# Autodesk Inventor assembly: Assembly7
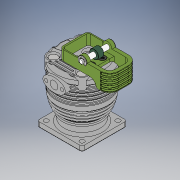
[picture p0: Inventor's stored thumbnail of the model, 180x180]
Saved by Autodesk Inventor 2018 (Build 220112000, 112)
## iProperties
Created: 2023-04-25
Part Number: Assembly7
Document SubType Name: Assembly
Designer: Habib Mohamed
Author: Habib Mohamed
## Documents named in this file (13)
- D:\Inventor\My projects\Rotary Engine\Assembly\Assembly7.iam
- Cykinder SubAssembly.iam
- D:\Inventor\My projects\Rotary Engine\Component 13 (Cylinder Liner).ipt
- D:\Inventor\My projects\Rotary Engine\Component 22 (Cylinder Base Gasket).ipt
- D:\Inventor\My projects\Rotary Engine\Component 35(Cylinder Top Gasket).ipt
- D:\Inventor\My projects\Rotary Engine\Component 50(Cylinder Head).ipt
- D:\Inventor\My projects\Rotary Engine\Component 49(Cylinder).ipt
- D:\Inventor\My projects\Rotary Engine\Component 25 (Rocker Arm Axle).ipt
- D:\Inventor\My projects\Rotary Engine\Component 36(Rocker Arm Bracket).ipt
- D:\Inventor\My projects\Rotary Engine\Component 14 (Spacer Sleeve).ipt
- C:\Users\Habib Mohamed\Documents\Inventor\Content Center Files\R2018\en-US\DIN EN ISO 4014\DIN EN ISO 4014 - M4 x 25.ipt
- C:\Users\Habib Mohamed\Documents\Inventor\Content Center Files\R2018\en-US\ISO 7046-1 Z(1)\ISO 7046-1 - M3 x 10 - 4.8 - Z - ISO.ipt
- C:\Users\Habib Mohamed\Documents\Inventor\Content Center Files\R2018\en-US\DIN 6799\DIN 6799 - 3.2 4.ipt
## Components (16 placed, 11 different names)
1. Component 13 (Cylinder Liner):1 — Mate:7, Mate:8, Mate:9, Mate:12
2. Component 22 (Cylinder Base Gasket):1 — Mate:11, Mate:12, Mate:13
3. Component 35(Cylinder Top Gasket):1 — Mate:6, Mate:9
4. Component 50(Cylinder Head):1 — Mate:4, Mate:5, Mate:10, Mate:15, Mate:17, Mate:19, Mate:21, Mate:22, Mate:23, Mate:24
5. Component 49(Cylinder):1 — Mate:1, Mate:2, Mate:3, Mate:4, Mate:5, Mate:6, Mate:7, Mate:8, Mate:10, Mate:11, Mate:13, Mate:14, Mate:16, Mate:18, Mate:20
6. Component 25 (Rocker Arm Axle):1 — Mate:25, Mate:26, Mate:27, Mate:31, Mate:33
7. Component 36(Rocker Arm Bracket):1 — Mate:22, Mate:23, Mate:24, Mate:26, Mate:27, Mate:28, Mate:29, Mate:30, Mate:32, Mate:34
8. Component 14 (Spacer Sleeve):1 — Mate:25, Mate:28
9. DIN EN ISO 4014 M4 x 25:1 — Mate:14, Mate:15
10. DIN EN ISO 4014 M4 x 25:2 — Mate:16, Mate:17
11. DIN EN ISO 4014 M4 x 25:3 — Mate:18, Mate:19
12. DIN EN ISO 4014 M4 x 25:4 — Mate:20, Mate:21
13. ISO 7046-1 Z M3 x 10 - 4.8 - Z:1 — Mate:29
14. ISO 7046-1 Z M3 x 10 - 4.8 - Z:2 — Mate:30
15. DIN 6799 3.2:1 — Mate:31, Mate:32
16. DIN 6799 3.2:2 — Mate:33, Mate:34
## Relationships (34: Mate 34)
- Mate:1: Component 49(Cylinder):1
- Mate:2: Component 49(Cylinder):1
- Mate:3: Component 49(Cylinder):1
- Mate:4: Component 50(Cylinder Head):1 ↔ Component 49(Cylinder):1
- Mate:5: Component 50(Cylinder Head):1 ↔ Component 49(Cylinder):1
- Mate:6: Component 35(Cylinder Top Gasket):1 ↔ Component 49(Cylinder):1
- Mate:7: Component 13 (Cylinder Liner):1 ↔ Component 49(Cylinder):1
- Mate:8: Component 13 (Cylinder Liner):1 ↔ Component 49(Cylinder):1
- Mate:9: Component 13 (Cylinder Liner):1 ↔ Component 35(Cylinder Top Gasket):1
- Mate:10: Component 50(Cylinder Head):1 ↔ Component 49(Cylinder):1
- Mate:11: Component 22 (Cylinder Base Gasket):1 ↔ Component 49(Cylinder):1
- Mate:12: Component 13 (Cylinder Liner):1 ↔ Component 22 (Cylinder Base Gasket):1
- Mate:13: Component 22 (Cylinder Base Gasket):1 ↔ Component 49(Cylinder):1
- Mate:14: Component 49(Cylinder):1 ↔ DIN EN ISO 4014 M4 x 25:1
- Mate:15: Component 50(Cylinder Head):1 ↔ DIN EN ISO 4014 M4 x 25:1
- Mate:16: Component 49(Cylinder):1 ↔ DIN EN ISO 4014 M4 x 25:2
- Mate:17: Component 50(Cylinder Head):1 ↔ DIN EN ISO 4014 M4 x 25:2
- Mate:18: Component 49(Cylinder):1 ↔ DIN EN ISO 4014 M4 x 25:3
- Mate:19: Component 50(Cylinder Head):1 ↔ DIN EN ISO 4014 M4 x 25:3
- Mate:20: Component 49(Cylinder):1 ↔ DIN EN ISO 4014 M4 x 25:4
- Mate:21: Component 50(Cylinder Head):1 ↔ DIN EN ISO 4014 M4 x 25:4
- Mate:22: Component 50(Cylinder Head):1 ↔ Component 36(Rocker Arm Bracket):1
- Mate:23: Component 50(Cylinder Head):1 ↔ Component 36(Rocker Arm Bracket):1
- Mate:24: Component 50(Cylinder Head):1 ↔ Component 36(Rocker Arm Bracket):1
- Mate:25: Component 25 (Rocker Arm Axle):1 ↔ Component 14 (Spacer Sleeve):1
- Mate:26: Component 25 (Rocker Arm Axle):1 ↔ Component 36(Rocker Arm Bracket):1
- Mate:27: Component 25 (Rocker Arm Axle):1 ↔ Component 36(Rocker Arm Bracket):1
- Mate:28: Component 36(Rocker Arm Bracket):1 ↔ Component 14 (Spacer Sleeve):1
- Mate:29: Component 36(Rocker Arm Bracket):1 ↔ ISO 7046-1 Z M3 x 10 - 4.8 - Z:1
- Mate:30: Component 36(Rocker Arm Bracket):1 ↔ ISO 7046-1 Z M3 x 10 - 4.8 - Z:2
- Mate:31: Component 25 (Rocker Arm Axle):1 ↔ DIN 6799 3.2:1
- Mate:32: Component 36(Rocker Arm Bracket):1 ↔ DIN 6799 3.2:1
- Mate:33: Component 25 (Rocker Arm Axle):1 ↔ DIN 6799 3.2:2
- Mate:34: Component 36(Rocker Arm Bracket):1 ↔ DIN 6799 3.2:2
